# Autodesk Inventor assembly: Vial Carousel
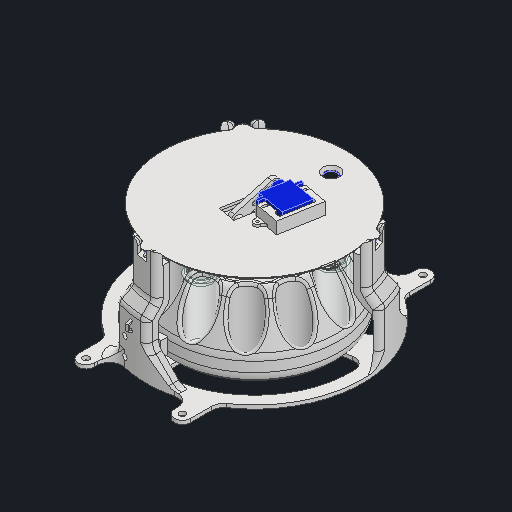
[picture p0: Inventor's stored thumbnail of the model, 512x512]
Saved by Autodesk Inventor 2025.1 (Build 291241000, 241)
## iProperties
Created: 2025-02-21
Part Number: Vial Carousel
Document SubType Name: Assembly
Designer: jerem
Author: jerem
## Documents named in this file (17)
- C:\Users\jerem\Documents\GitHub\Perovskite-Automated-Synthesis-System\CAD\vial carousel\Vial Carousel.iam
- C:\Users\jerem\Documents\GitHub\Perovskite-Automated-Synthesis-System\CAD\Non 3D Printed Parts\Motors and Servos\NEMA17 Stepper Motor - 26 mm.ipt
- C:\Users\jerem\Documents\GitHub\Perovskite-Automated-Synthesis-System\CAD\vial carousel\Vial Holder.ipt
- C:\Users\jerem\Documents\GitHub\Perovskite-Automated-Synthesis-System\CAD\Non 3D Printed Parts\Vial.ipt
- C:\Users\jerem\Documents\GitHub\Perovskite-Automated-Synthesis-System\CAD\vial carousel\Motor Mount.ipt
- C:\Users\jerem\Documents\GitHub\Perovskite-Automated-Synthesis-System\CAD\vial carousel\Shaft Collar.ipt
- C:\Users\jerem\Documents\GitHub\Perovskite-Automated-Synthesis-System\CAD\vial carousel\Vial Cover.ipt
- C:\Users\jerem\Documents\GitHub\Perovskite-Automated-Synthesis-System\CAD\Non 3D Printed Parts\Limit Switch.ipt
- C:\Users\jerem\Documents\GitHub\Perovskite-Automated-Synthesis-System\CAD\Non 3D Printed Parts\Bearings\5x5x11bearing.ipt
- C:\Users\jerem\Documents\GitHub\Perovskite-Automated-Synthesis-System\CAD\vial carousel\Bearing Grip.ipt
- C:\Users\jerem\Documents\GitHub\Perovskite-Automated-Synthesis-System\CAD\vial carousel\Bearing Mount.ipt
- C:\Users\jerem\Documents\GitHub\Perovskite-Automated-Synthesis-System\CAD\Non 3D Printed Parts\Motors and Servos\SG90 Servo.ipt
- C:\Users\jerem\Documents\GitHub\Perovskite-Automated-Synthesis-System\CAD\Non 3D Printed Parts\Motors and Servos\HalfServoArm.ipt
- C:\Users\jerem\Documents\GitHub\Perovskite-Automated-Synthesis-System\CAD\vial carousel\Servo Arm.ipt
- C:\Users\jerem\Documents\GitHub\Perovskite-Automated-Synthesis-System\CAD\vial carousel\Link.ipt
- C:\Users\jerem\Documents\GitHub\Perovskite-Automated-Synthesis-System\CAD\vial carousel\Servo Holder.ipt
- C:\Users\jerem\Documents\GitHub\Perovskite-Automated-Synthesis-System\CAD\Non 3D Printed Parts\Screws\M2x8.ipt
## Components (22 placed, 16 different names)
1. NEMA17 Stepper Motor - 26 mm:1 — Mate:7, Mate:8, Mate:9, Mate:11, Mate:19, Mate:22
2. Vial Holder:1 — Mate:1, Mate:2, Mate:3, Mate:4, Mate:5, Mate:6, Mate:19, Mate:20, Mate:23, Mate:24, Mate:25, Mate:26, Mate:56, Mate:57, Mate:58, Mate:59
3. Vial:1 — Mate:4, Mate:5
4. Vial:2 — Mate:3, Mate:6
5. Vial:3 — Mate:1, Mate:2
6. Motor Mount:1 — Mate:7, Mate:8, Mate:9, Mate:28, Mate:29, Mate:30, Mate:66
7. Shaft Collar:1 — Mate:11, Mate:20, Mate:22, Mate:23, Mate:32, Mate:33, Mate:34
8. Vial Cover:1 — Mate:24, Mate:37, Angle:2, Mate:52, Mate:53, Mate:66
9. Vial:4 — Mate:25, Mate:26
10. Limit Switch:1 — Mate:28, Mate:29, Mate:30
11. 5x5x11bearing:1 — Mate:31, Mate:35, Mate:36, Mate:65
12. Bearing Grip:1 — Mate:31, Mate:35, Angle:1, Mate:47, Mate:60
13. Bearing Mount:1 — Mate:32, Mate:33, Mate:34, Mate:36, Mate:65
14. SG90 Servo:1 — Mate:37, Angle:1, Mate:38, Mate:39, Angle:2, Mate:49, Mate:63, Mate:64
15. HalfServoArm:1 — Mate:38, Mate:39, Mate:41, Mate:42, Flush:44
16. Servo Arm:1 — Mate:41, Mate:42, Flush:44, Mate:46
17. Link:1 — Mate:46, Mate:47, Mate:60, Mate:61, Mate:62
18. Servo Holder:1 — Mate:49, Mate:52, Mate:53, Mate:63, Mate:64
19. M2x8:1 — Mate:61
20. M2x8:2 — Mate:62
21. Vial:5 — Mate:56, Mate:57
22. Vial:6 — Mate:58, Mate:59
## Relationships (50: Mate 47, Angle 2, Flush 1)
- Mate:1: Vial Holder:1 ↔ Vial:3
- Mate:2: Vial Holder:1 ↔ Vial:3
- Mate:3: Vial Holder:1 ↔ Vial:2
- Mate:4: Vial Holder:1 ↔ Vial:1
- Mate:5: Vial Holder:1 ↔ Vial:1
- Mate:6: Vial Holder:1 ↔ Vial:2
- Mate:7: NEMA17 Stepper Motor - 26 mm:1 ↔ Motor Mount:1
- Mate:8: NEMA17 Stepper Motor - 26 mm:1 ↔ Motor Mount:1
- Mate:9: NEMA17 Stepper Motor - 26 mm:1 ↔ Motor Mount:1
- Mate:11: NEMA17 Stepper Motor - 26 mm:1 ↔ Shaft Collar:1
- Mate:19: NEMA17 Stepper Motor - 26 mm:1 ↔ Vial Holder:1
- Mate:20: Vial Holder:1 ↔ Shaft Collar:1
- Mate:22: NEMA17 Stepper Motor - 26 mm:1 ↔ Shaft Collar:1
- Mate:23: Vial Holder:1 ↔ Shaft Collar:1
- Mate:24: Vial Holder:1 ↔ Vial Cover:1
- Mate:25: Vial Holder:1 ↔ Vial:4
- Mate:26: Vial Holder:1 ↔ Vial:4
- Mate:28: Motor Mount:1 ↔ Limit Switch:1
- Mate:29: Motor Mount:1 ↔ Limit Switch:1
- Mate:30: Motor Mount:1 ↔ Limit Switch:1
- Mate:31: 5x5x11bearing:1 ↔ Bearing Grip:1
- Mate:32: Shaft Collar:1 ↔ Bearing Mount:1
- Mate:33: Shaft Collar:1 ↔ Bearing Mount:1
- Mate:34: Shaft Collar:1 ↔ Bearing Mount:1
- Mate:35: 5x5x11bearing:1 ↔ Bearing Grip:1
- Mate:36: 5x5x11bearing:1 ↔ Bearing Mount:1
- Mate:37: Vial Cover:1 ↔ SG90 Servo:1
- Angle:1 (0 deg): Bearing Grip:1 ↔ SG90 Servo:1
- Mate:38: SG90 Servo:1 ↔ HalfServoArm:1
- Mate:39: SG90 Servo:1 ↔ HalfServoArm:1
- Angle:2 (0 deg): Vial Cover:1 ↔ SG90 Servo:1
- Mate:41: HalfServoArm:1 ↔ Servo Arm:1
- Mate:42: HalfServoArm:1 ↔ Servo Arm:1
- Flush:44: HalfServoArm:1 ↔ Servo Arm:1
- Mate:46: Servo Arm:1 ↔ Link:1
- Mate:47: Bearing Grip:1 ↔ Link:1
- Mate:49: SG90 Servo:1 ↔ Servo Holder:1
- Mate:52: Vial Cover:1 ↔ Servo Holder:1
- Mate:53: Vial Cover:1 ↔ Servo Holder:1
- Mate:56: Vial Holder:1 ↔ Vial:5
- Mate:57: Vial Holder:1 ↔ Vial:5
- Mate:58: Vial Holder:1 ↔ Vial:6
- Mate:59: Vial Holder:1 ↔ Vial:6
- Mate:60: Bearing Grip:1 ↔ Link:1
- Mate:61: Link:1 ↔ M2x8:1
- Mate:62: Link:1 ↔ M2x8:2
- Mate:63: SG90 Servo:1 ↔ Servo Holder:1
- Mate:64: SG90 Servo:1 ↔ Servo Holder:1
- Mate:65: 5x5x11bearing:1 ↔ Bearing Mount:1
- Mate:66: Motor Mount:1 ↔ Vial Cover:1
